# Autodesk Inventor assembly: Rear_Train
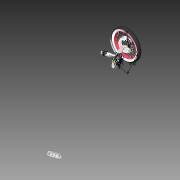
[picture p0: Inventor's stored thumbnail of the model, 180x180]
Saved by Autodesk Inventor 2016 (Build 200138000, 138)
## iProperties
Created: 2015-04-04
Part Number: Rear_Train
Document SubType Name: Assembly
Designer: Yann
Author: Yann
## Documents named in this file (6)
- C:\Users\Yann\Documents\GitHub\Bikair_CAD\Source\Rear_Train\Rear_Train.iam
- C:\Users\Yann\Documents\GitHub\Bikair_CAD\Source\Rear_Train\Swing_Arm.iam
- C:\Users\Yann\Documents\GitHub\Bikair_CAD\Source\Rear_Train\Suspension\ShockAbsorber.iam
- C:\Users\Yann\Documents\GitHub\Bikair_CAD\Source\Front_Train\Wheel_spokes\Wheel_spokes.iam
- C:\Users\Yann\Documents\GitHub\Bikair_CAD\Source\Rear_Train\REAR FENDER-VAL.ipt
- C:\Users\Yann\Documents\GitHub\Bikair_CAD\Source\Rear_Train\Motor\Motor.iam
## Components (5 placed, 5 different names)
1. Wheel_spokes:1 [sub-assembly] — Mate:9, Flush:11
2. Swing_Arm:1 [sub-assembly] — Mate:3, Flush:2, Mate:7
3. ShockAbsorber:1 [sub-assembly] — Mate:7, Mate:13
4. REAR FENDER-VAL:1 — Mate:12
5. Motor:1 [sub-assembly] — Mate:14, Mate:15
## Relationships (9: Mate 7, Flush 2)
- Mate:3: Swing_Arm:1
- Flush:2: Swing_Arm:1
- Mate:7: Swing_Arm:1 ↔ ShockAbsorber:1
- Mate:9: Wheel_spokes:1
- Flush:11: Wheel_spokes:1
- Mate:12: REAR FENDER-VAL:1
- Mate:13: ShockAbsorber:1
- Mate:14: Motor:1
- Mate:15: Motor:1
